# Autodesk Inventor assembly: carriage
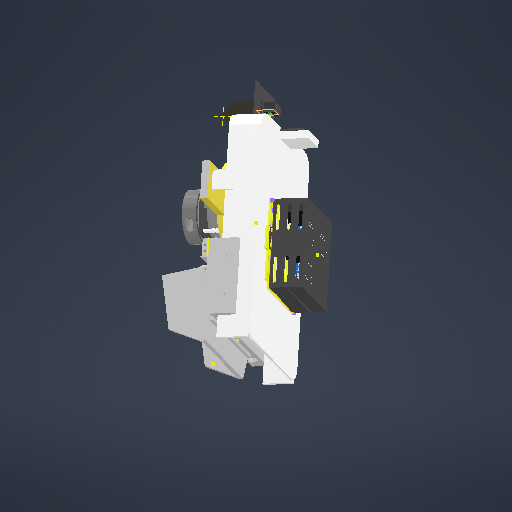
[picture p0: Inventor's stored thumbnail of the model, 512x512]
Saved by Autodesk Inventor 2027 (Build 310192000, 192)
## iProperties
Created: 2026-06-28
Part Number: carriage
Document SubType Name: Assembly
Designer: uchiha
Author: uchiha
## Documents named in this file (14)
- C:\Users\uchiha\Desktop\New folder\designdj\parts\rocker-bogie-mechanism-mars-rover-1.snapshot.9\carriage.iam
- C:\Users\uchiha\Desktop\New folder\designdj\partoscrew2.5mm.ipt
- C:\Users\uchiha\Desktop\New folder\designdj\parts\rocker-bogie-mechanism-mars-rover-1.snapshot.9\base\base.ipt
- C:\Users\uchiha\Desktop\New folder\designdj\parts\parts\rplidar-a1-holder-1.snapshot.2\12\RP-lidar-A1.igs.iam
- C:\Users\uchiha\Desktop\New folder\designdj\parts\arduino-uno-r3-8.snapshot.2\Arduino Uno\Arduino Uno.ipt
- C:\Users\uchiha\Desktop\New folder\designdj\parts\parts\boitier-raspberry-pi-4-2.snapshot.2 (1)\Assemblage1\Assemblage1.iam
- C:\Users\uchiha\Desktop\New folder\designdj\New folder\MOTOR DRIVER ASSEMBLY.iam
- C:\Users\uchiha\Desktop\New folder\designdj\CameraPanTiltFiles\CameraPanTiltAssy.iam
- C:\Users\uchiha\Documents\Inventor\Content Center Files\R2027\en-US\AS 1110\AS 1110 - M1.6 x 6.ipt
- C:\Users\uchiha\Desktop\New folder\designdj\auraclerobot\sensormounts\lidarholder - Copy.ipt
- C:\Users\uchiha\Desktop\New folder\designdj\auraclerobot\motordriverholder.ipt
- C:\Users\uchiha\Desktop\New folder\designdj\rackpinion.ipt.iam
- C:\Users\uchiha\Desktop\New folder\designdj\auraclerobot\mounts\motordriverholder\motordriverholder.ipt
- rackpinion.ipt
## Components (18 placed, 11 different names)
1. partoscrew2.5mm:1
2. partoscrew2.5mm:2
3. partoscrew2.5mm:3
4. partoscrew2.5mm:4
5. base:1 — Mate:12, Mate:13, Mate:14, Mate:15, Mate:16, Mate:17, Mate:18, Mate:19, Mate:20, Mate:21, Mate:22, Mate:23, Mate:24, Mate:25, Mate:26, Mate:27, Flush:1, Flush:2, Flush:3, Mate:29, Mate:32, Mate:33, Mate:35, Mate:36, Flush:4, Mate:38
6. RP-lidar-A1.igs:1 [sub-assembly] — Mate:30, Mate:31
7. Arduino Uno:2 — Mate:12, Mate:13, Mate:14, Mate:15
8. Assemblage1:1 [sub-assembly] — Mate:16, Mate:17, Mate:18, Mate:19, Mate:20
9. MOTOR DRIVER ASSEMBLY:1 [sub-assembly] — Mate:21, Mate:22, Mate:23, Mate:34, Mate:37, Mate:38, Mate:39, Mate:40, Mate:41
10. CameraPanTiltAssy:1 [sub-assembly] — Mate:24, Mate:25, Mate:26, Insert:1, Insert:2, Insert:3, Insert:4, Mate:27
11. AS 1110 - Metric M1.6 x 6:1 — Insert:1
12. AS 1110 - Metric M1.6 x 6:2 — Insert:2
13. AS 1110 - Metric M1.6 x 6:3 — Insert:3
14. AS 1110 - Metric M1.6 x 6:4 — Insert:4
15. lidarholder - Copy:1 — Mate:29, Mate:30, Mate:31
16. motordriverholder:1 — Mate:32, Mate:33, Mate:34
17. rackpinion.ipt:1 [sub-assembly] — Mate:35, Mate:36
18. motordriverholder:2 — Mate:37, Mate:39, Mate:40, Mate:41
## Relationships (37: Mate 29, Insert 4, Flush 4)
- Mate:12: base:1 ↔ Arduino Uno:2
- Mate:13: base:1 ↔ Arduino Uno:2
- Mate:14: base:1 ↔ Arduino Uno:2
- Mate:15: base:1 ↔ Arduino Uno:2
- Mate:16: base:1 ↔ Assemblage1:1
- Mate:17: base:1 ↔ Assemblage1:1
- Mate:18: base:1 ↔ Assemblage1:1
- Mate:19: base:1 ↔ Assemblage1:1
- Mate:20: base:1 ↔ Assemblage1:1
- Mate:21 (5 mm): base:1 ↔ MOTOR DRIVER ASSEMBLY:1
- Mate:22: base:1 ↔ MOTOR DRIVER ASSEMBLY:1
- Mate:23: base:1 ↔ MOTOR DRIVER ASSEMBLY:1
- Mate:24: base:1 ↔ CameraPanTiltAssy:1
- Mate:25: base:1 ↔ CameraPanTiltAssy:1
- Mate:26: base:1 ↔ CameraPanTiltAssy:1
- Insert:1: CameraPanTiltAssy:1 ↔ AS 1110 - Metric M1.6 x 6:1
- Insert:2: CameraPanTiltAssy:1 ↔ AS 1110 - Metric M1.6 x 6:2
- Insert:3: CameraPanTiltAssy:1 ↔ AS 1110 - Metric M1.6 x 6:3
- Insert:4: CameraPanTiltAssy:1 ↔ AS 1110 - Metric M1.6 x 6:4
- Mate:27: base:1 ↔ CameraPanTiltAssy:1
- Flush:1: base:1
- Flush:2: base:1
- Flush:3: base:1
- Mate:29: base:1 ↔ lidarholder - Copy:1
- Mate:30: RP-lidar-A1.igs:1 ↔ lidarholder - Copy:1
- Mate:31: RP-lidar-A1.igs:1 ↔ lidarholder - Copy:1
- Mate:32: base:1 ↔ motordriverholder:1
- Mate:33: base:1 ↔ motordriverholder:1
- Mate:34: MOTOR DRIVER ASSEMBLY:1 ↔ motordriverholder:1
- Mate:35: base:1 ↔ rackpinion.ipt:1
- Mate:36: base:1 ↔ rackpinion.ipt:1
- Flush:4: base:1
- Mate:37: MOTOR DRIVER ASSEMBLY:1 ↔ motordriverholder:2
- Mate:38: base:1 ↔ MOTOR DRIVER ASSEMBLY:1
- Mate:39: MOTOR DRIVER ASSEMBLY:1 ↔ motordriverholder:2
- Mate:40: MOTOR DRIVER ASSEMBLY:1 ↔ motordriverholder:2
- Mate:41: MOTOR DRIVER ASSEMBLY:1 ↔ motordriverholder:2
